# Autodesk Inventor assembly: Main
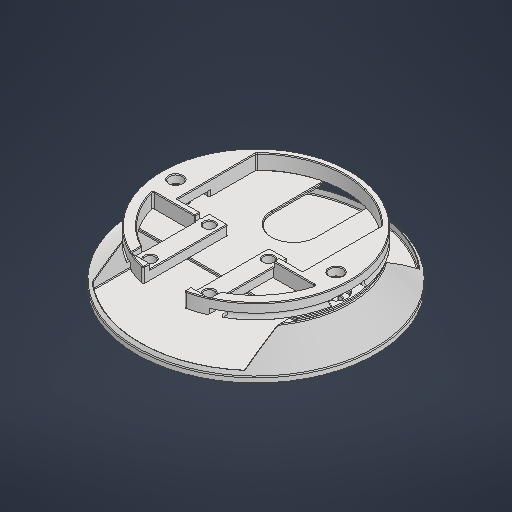
[picture p0: Inventor's stored thumbnail of the model, 512x512]
Saved by Autodesk Inventor 2026.1 (Build 301233020, 233B)
## iProperties
Created: 2025-09-16
Part Number: Main
Document SubType Name: Assembly
Designer: Administrator
Author: Administrator
## Documents named in this file (4)
- C:\Users\Administrator\Desktop\Doorbell\MCAD\Main.iam
- C:\Users\Administrator\Desktop\Doorbell\MCAD\Base.ipt
- C:\Users\Administrator\Desktop\Doorbell\MCAD\Battery Cover.ipt
- C:\Users\Administrator\Desktop\Doorbell\MCAD\Inner Superstructure.ipt
## Components (3 placed, 3 different names)
1. Base:1 — Mate:1, Mate:2, Mate:3, Mate:5, Mate:6
2. Battery Cover:1 — Mate:1, Mate:2, Mate:3, Mate:4
3. Inner Superstructure:1 — Mate:4, Mate:5, Mate:6
## Relationships (6: Mate 6)
- Mate:1: Base:1 ↔ Battery Cover:1
- Mate:2: Base:1 ↔ Battery Cover:1
- Mate:3: Base:1 ↔ Battery Cover:1
- Mate:4 (1 mm): Battery Cover:1 ↔ Inner Superstructure:1
- Mate:5: Base:1 ↔ Inner Superstructure:1
- Mate:6: Base:1 ↔ Inner Superstructure:1
